# Autodesk Inventor assembly: COSI_MINI_V1
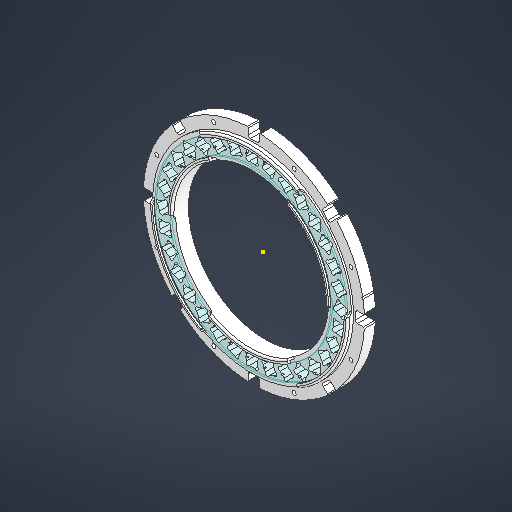
[picture p0: Inventor's stored thumbnail of the model, 512x512]
Saved by Autodesk Inventor 2026.1 (Build 301233020, 233B)
## iProperties
Created: 2023-07-27
Part Number: COSI_MINI_V1
Document SubType Name: Assembly
Designer: Joshua Harper
Author: Joshua Harper
## Documents named in this file (18)
- C:\Users\Carla Fernandez\Documents\GitHub\OSII_MINI_V2\CAD MODELS_screw_on\COSI_MINI_V2.iam
- C:\Users\Carla Fernandez\Documents\GitHub\OSII_MINI_V2\CAD MODELS_screw_on\Ring_0.ipt
- C:\Users\Carla Fernandez\Documents\GitHub\OSII_MINI_V2\CAD MODELS_screw_on\Ring_1.ipt
- C:\Users\Carla Fernandez\Documents\GitHub\OSII_MINI_V2\CAD MODELS_screw_on\Ring_2.ipt
- C:\Users\Carla Fernandez\Documents\GitHub\OSII_MINI_V2\CAD MODELS_screw_on\Ring_3.ipt
- C:\Users\Carla Fernandez\Documents\GitHub\OSII_MINI_V2\CAD MODELS_screw_on\Ring_4.ipt
- C:\Users\Carla Fernandez\Documents\GitHub\OSII_MINI_V2\CAD MODELS_screw_on\M4_threaded_brass.ipt
- C:\Users\Carla Fernandez\Documents\GitHub\OSII_MINI_V2\CAD MODELS_screw_on\Locating_bar_V2.ipt
- C:\Users\Carla Fernandez\Documents\GitHub\OSII_MINI_V2\CAD MODELS_screw_on\93187A150_NO THREADS_Brass Thin Hex Nut.ipt
- C:\Users\Carla Fernandez\Documents\GitHub\OSII_MINI_V2\CAD MODELS_screw_on\98691A114_General Purpose Brass Washer.ipt
- C:\Users\Carla Fernandez\Documents\GitHub\OSII_MINI_V2\CAD MODELS_screw_on\94500A283_NO THREADS_316 Stainless Steel Button Head Hex Drive Screws.ipt
- C:\Users\Carla Fernandez\Documents\GitHub\OSII_MINI_V2\CAD MODELS_screw_on\94500A283_NO THREADS_316 Stainless Steel Button Head Hex Drive Screws_MIR.ipt
- C:\Users\Carla Fernandez\Documents\GitHub\OSII_MINI_V2\CAD MODELS_screw_on\Lid_A.ipt
- C:\Users\Carla Fernandez\Documents\GitHub\OSII_MINI_V2\CAD MODELS_screw_on\Lid_B.ipt
- C:\Users\Carla Fernandez\Documents\GitHub\OSII_MINI_V2\CAD MODELS_screw_on\Shim_Assem_V4.iam
- C:\Users\Carla Fernandez\Documents\GitHub\OSII_MINI_V2\CAD MODELS_screw_on\shim_cartridge_V3.ipt
- C:\Users\Carla Fernandez\Documents\GitHub\OSII_MINI_V2\CAD MODELS_screw_on\shim_peg_V3.ipt
- C:\Users\Carla Fernandez\Documents\GitHub\OSII_MINI_V2\CAD MODELS_screw_on\Gradient_coil.ipt
## Components (23 placed, 17 different names)
1. Ring_0:1 — Mate:4, Mate:5, Mate:16, Mate:70, Mate:71, Flush:3, Flush:4, Flush:5, Flush:6, Mate:82, Mate:83, Mate:84, Mate:86, Mate:87, Mate:88, Mate:89
2. Ring_1:1 — Mate:5, Mate:17, Flush:3, Mate:82
3. Ring_1:2 — Mate:3, Mate:4, Mate:10, Mate:16, Mate:87
4. Ring_2:1 — Mate:6, Mate:17, Flush:4, Mate:83
5. Ring_2:2 — Mate:2, Mate:3, Mate:9, Mate:10, Mate:86
6. Ring_3:1 — Mate:6, Mate:7, Flush:5, Mate:84
7. Ring_3:2 — Mate:1, Mate:2, Mate:8, Mate:9, Mate:36, Mate:88
8. Ring_4:1 — Mate:7, Flush:6, Mate:72, Mate:73
9. Ring_4:2 — Mate:1, Mate:8, Mate:26, Mate:35, Mate:62, Mate:63, Mate:68, Mate:89
10. Locating_bar_V2:1 — Mate:35, Mate:36, Mate:69
11. 98691A114_General Purpose Brass Washer:2 — Mate:63, Mate:66
12. 98691A114_General Purpose Brass Washer:1 — Mate:62, Mate:67
13. 93187A150_NO THREADS_Brass Thin Hex Nut:2 — Mate:66
14. 93187A150_NO THREADS_Brass Thin Hex Nut:1 — Mate:67
15. 94500A283_NO THREADS_316 Stainless Steel Button Head Hex Drive Screws:1 — Mate:68, Mate:69
16. Lid_A:1 — Mate:70, Mate:71
17. Lid_B:1
18. 94500A283_NO THREADS_316 Stainless Steel Button Head Hex Drive Screws_MIR:1 — Mate:72, Mate:73
19. M4_threaded_brass:1 — Mate:26
20. Shim_Assem_V4:1 [sub-assembly] — Mate:78, Mate:80, Mate:81
21. shim_cartridge_V3:1 — Mate:80, Mate:81
22. shim_peg_V3:1 — Mate:78
23. Gradient_coil:1 — Flush:7
## Relationships (40: Mate 35, Flush 5)
- Mate:1 (12 mm): Ring_3:2 ↔ Ring_4:2
- Mate:2 (12 mm): Ring_2:2 ↔ Ring_3:2
- Mate:3 (12 mm): Ring_1:2 ↔ Ring_2:2
- Mate:4 (12 mm): Ring_0:1 ↔ Ring_1:2
- Mate:5 (12 mm): Ring_0:1 ↔ Ring_1:1
- Mate:6 (12 mm): Ring_2:1 ↔ Ring_3:1
- Mate:7 (12 mm): Ring_3:1 ↔ Ring_4:1
- Mate:8: Ring_3:2 ↔ Ring_4:2
- Mate:9: Ring_2:2 ↔ Ring_3:2
- Mate:10: Ring_1:2 ↔ Ring_2:2
- Mate:16: Ring_0:1 ↔ Ring_1:2
- Mate:17 (12 mm): Ring_1:1 ↔ Ring_2:1
- Mate:26: Ring_4:2 ↔ M4_threaded_brass:1
- Mate:35: Ring_4:2 ↔ Locating_bar_V2:1
- Mate:36: Ring_3:2 ↔ Locating_bar_V2:1
- Mate:62: Ring_4:2 ↔ 98691A114_General Purpose Brass Washer:1
- Mate:63: Ring_4:2 ↔ 98691A114_General Purpose Brass Washer:2
- Mate:66: 98691A114_General Purpose Brass Washer:2 ↔ 93187A150_NO THREADS_Brass Thin Hex Nut:2
- Mate:67: 98691A114_General Purpose Brass Washer:1 ↔ 93187A150_NO THREADS_Brass Thin Hex Nut:1
- Mate:68: Ring_4:2 ↔ 94500A283_NO THREADS_316 Stainless Steel Button Head Hex Drive Screws:1
- Mate:69: Locating_bar_V2:1 ↔ 94500A283_NO THREADS_316 Stainless Steel Button Head Hex Drive Screws:1
- Mate:70: Ring_0:1 ↔ Lid_A:1
- Mate:71: Ring_0:1 ↔ Lid_A:1
- Flush:3: Ring_0:1 ↔ Ring_1:1
- Flush:4: Ring_0:1 ↔ Ring_2:1
- Flush:5: Ring_0:1 ↔ Ring_3:1
- Flush:6: Ring_0:1 ↔ Ring_4:1
- Mate:72: Ring_4:1 ↔ 94500A283_NO THREADS_316 Stainless Steel Button Head Hex Drive Screws_MIR:1
- Mate:73: Ring_4:1 ↔ 94500A283_NO THREADS_316 Stainless Steel Button Head Hex Drive Screws_MIR:1
- Mate:78: Shim_Assem_V4:1 ↔ shim_peg_V3:1
- Mate:80: Shim_Assem_V4:1 ↔ shim_cartridge_V3:1
- Mate:81: Shim_Assem_V4:1 ↔ shim_cartridge_V3:1
- Mate:82: Ring_0:1 ↔ Ring_1:1
- Mate:83: Ring_0:1 ↔ Ring_2:1
- Mate:84: Ring_0:1 ↔ Ring_3:1
- Mate:86: Ring_0:1 ↔ Ring_2:2
- Mate:87: Ring_0:1 ↔ Ring_1:2
- Mate:88: Ring_0:1 ↔ Ring_3:2
- Mate:89: Ring_0:1 ↔ Ring_4:2
- Flush:7: Gradient_coil:1
## Named parameters: r_space = 12 mm
